# Autodesk Inventor assembly: minisumo_złożenie
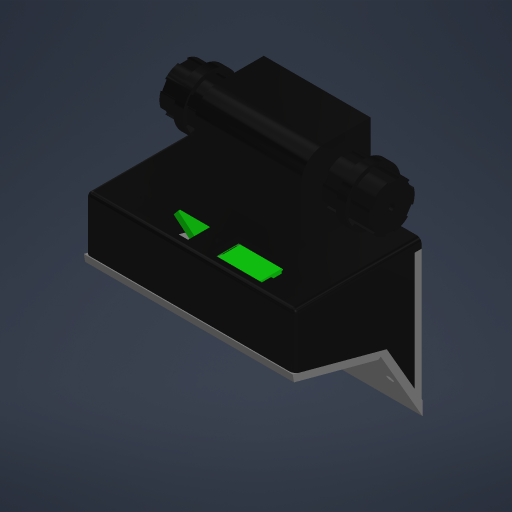
[picture p0: Inventor's stored thumbnail of the model, 512x512]
Saved by Autodesk Inventor 2023.4 (Build 274418000, 418)
## iProperties
Created: 2025-10-31
Part Number: minisumo_złożenie
Document SubType Name: Assembly
Designer: Jakub Borsukiewicz
Author: Jakub Borsukiewicz
## Documents named in this file (7)
- C:\Users\KUBA\Desktop\AiR\Semestr 5\ARES-minisumo-robot\mechanics\minisumo_złożenie.iam
- C:\Users\KUBA\Desktop\AiR\Semestr 5\ARES-minisumo-robot\mechanics\koło.ipt
- C:\Users\KUBA\Desktop\AiR\Semestr 5\ARES-minisumo-robot\mechanics\obciążenie_dół.ipt
- C:\Users\KUBA\Desktop\AiR\Semestr 5\ARES-minisumo-robot\mechanics\obudowa_robota.ipt
- C:\Users\KUBA\Desktop\AiR\Semestr 5\ARES-minisumo-robot\mechanics\pług_część1.ipt
- C:\Users\KUBA\Desktop\AiR\Semestr 5\ARES-minisumo-robot\mechanics\pług_część2.ipt
- C:\Users\KUBA\Desktop\AiR\Semestr 5\ARES-minisumo-robot\mechanics\płytka_pcb.ipt
## Components (7 placed, 6 different names)
1. koło:1 — Obrotowe:1
2. obciążenie_dół:1 — Zestawiające:1, Zestawiające:2
3. obudowa_robota:1 — Zestawiające:1, Zestawiające:2, Zestawiające:3, Zestawiające:4, Zestawiające:5, Zestawiające:6, Obrotowe:1, Obrotowe:2, Wstawiające:1, Wstawiające:2
4. pług_część1:1 — Zestawiające:3, Zestawiające:4
5. pług_część2:1 — Zestawiające:5, Zestawiające:6
6. koło:2 — Obrotowe:2
7. płytka_pcb:1 — Wstawiające:1, Wstawiające:2
## Relationships (10: Mate 6, RevoluteJoint 2, Insert 2)
- Zestawiające:1 [Mate]: obciążenie_dół:1 ↔ obudowa_robota:1
- Zestawiające:2 [Mate]: obciążenie_dół:1 ↔ obudowa_robota:1
- Zestawiające:3 [Mate]: obudowa_robota:1 ↔ pług_część1:1
- Zestawiające:4 [Mate]: obudowa_robota:1 ↔ pług_część1:1
- Zestawiające:5 [Mate]: obudowa_robota:1 ↔ pług_część2:1
- Zestawiające:6 [Mate]: obudowa_robota:1 ↔ pług_część2:1
- Obrotowe:1 [RevoluteJoint] (2 mm): koło:1 ↔ obudowa_robota:1
- Obrotowe:2 [RevoluteJoint] (2 mm): obudowa_robota:1 ↔ koło:2
- Wstawiające:1 [Insert]: obudowa_robota:1 ↔ płytka_pcb:1
- Wstawiające:2 [Insert]: obudowa_robota:1 ↔ płytka_pcb:1
